# Autodesk Inventor assembly: CycloidalGearBoxAssemblyV2
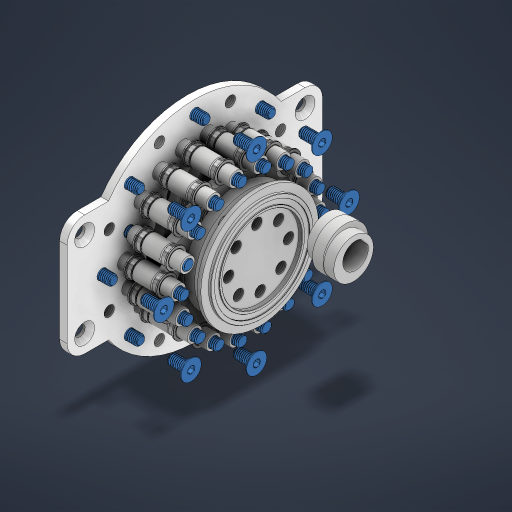
[picture p0: Inventor's stored thumbnail of the model, 512x512]
Saved by Autodesk Inventor 2024 (Build 280153000, 153)
## iProperties
Created: 2024-01-31
Part Number: CycloidalGearBoxAssemblyV2
Document SubType Name: Assembly
Designer: avsar
Author: avsar
## Documents named in this file (20)
- C:\Users\avsar\Documents\Inventor\RCR_Arm\Arm_V4\CycloidalGearBoxes\StageOneGearBox\CycloidalGearBoxAssemblyV2.iam
- C:\Users\avsar\Documents\Inventor\RCR_Arm\Arm_V4\CycloidalGearBoxes\StageOneGearBox\HousingFaceInput.ipt
- C:\Users\avsar\Documents\Inventor\RCR_Arm\Arm_V4\CycloidalGearBoxes\StageOneGearBox\HousingInputFaceSpacer.ipt
- C:\Users\avsar\Documents\Inventor\RCR_Arm\COTS\Motion\Bearings\Flanged Bearings\4x7x2.5mm Flanged Ball Bearing.ipt
- C:\Users\avsar\Documents\Inventor\RCR_Arm\Arm_V4\CycloidalGearBoxes\StageOneGearBox\RollerBearingShaft.ipt
- C:\Users\avsar\Documents\Inventor\RCR_Arm\Arm_V4\CycloidalGearBoxes\StageOneGearBox\EccentricBearingShaft.ipt
- C:\Users\avsar\Documents\Inventor\RCR_Arm\Arm_V4\CycloidalGearBoxes\StageOneGearBox\CycloidalDisk.ipt
- C:\Users\avsar\Documents\Inventor\RCR_Arm\COTS\Motion\Bearings\Standard Bearings\16mm ID x 22mm OD x 4mm Thickness Ball Bearing.ipt
- C:\Users\avsar\Documents\Inventor\RCR_Arm\Arm_V4\CycloidalGearBoxes\StageOneGearBox\OutputPlateSpacer.ipt
- C:\Users\avsar\Documents\Inventor\RCR_Arm\Arm_V4\CycloidalGearBoxes\StageOneGearBox\OutPutPlate.ipt
- C:\Users\avsar\Documents\Inventor\RCR_Arm\COTS\ISO Standard Hardware\Screws\Sockethead Screws\Buttonhead Screws\M4 x 0.7mm\(M4 x 0.7 x 18) Sockethead Buttonhead Screw.ipt
- C:\Users\avsar\Documents\Inventor\RCR_Arm\Arm_V4\CycloidalGearBoxes\StageOneGearBox\HousingLidSpacer.ipt
- C:\Users\avsar\Documents\Inventor\RCR_Arm\COTS\goBilda\Motion\Bearings\32mm ID Flanged Ball Bearing (39mm OD, 5mm Thickness).ipt
- C:\Users\avsar\Documents\Inventor\RCR_Arm\Arm_V4\CycloidalGearBoxes\StageOneGearBox\Gearbox_MainBody.ipt
- C:\Users\avsar\Documents\Inventor\RCR_Arm\Arm_V4\CycloidalGearBoxes\StageOneGearBox\HousingLid.ipt
- C:\Users\avsar\Documents\Inventor\RCR_Arm\Arm_V4\CycloidalGearBoxes\StageOneGearBox\InputSpacer.ipt
- C:\Users\avsar\Documents\Inventor\RCR_Arm\COTS\Motion\Bearings\Flanged Bearings\10x15x4mm Flanged Bearing.ipt
- C:\Users\avsar\Documents\Inventor\RCR_Arm\Arm_V4\CycloidalGearBoxes\StageOneGearBox\OutputBearingDistanceRing.ipt
- C:\Users\avsar\Documents\Inventor\RCR_Arm\COTS\ISO Standard Hardware\Screws\Sockethead Screws\Countersunk Screws\M4 x 0.7mm\(M4 x 0.7 x 8) Sockethead Countersunk Screw.ipt
- C:\Users\avsar\Documents\Inventor\RCR_Arm\Arm_V4\ArmStages\27mm_SandedScrew.ipt
## Components (168 placed, 19 different names)
1. HousingInputFaceSpacer:1 — Mate:3, Mate:4, Mate:305
2. 4x7x2.5mm Flanged Ball Bearing:1 — Mate:3, Mate:4, Mate:5, Mate:6, Mate:13
3. 4x7x2.5mm Flanged Ball Bearing:2 — Mate:7, Mate:8, Mate:108, Mate:109
4. RollerBearingShaft:1 — Mate:5, Mate:6, Mate:7, Mate:8, Mate:287
5. EccentricBearingShaft:1 — Mate:10, Mate:11, Mate:14, Mate:15, Mate:324
6. CycloidalDisk:1 — Flush:1, Mate:9, Mate:13, Mate:25, Tangent:1, Mate:32, Mate:33, Mate:34, Mate:35, Mate:36, Tangent:8, Tangent:9, Tangent:10, Tangent:11, Tangent:12, Tangent:13
7. 16mm ID x 22mm OD x 4mm Thickness Ball Bearing:1 — Flush:1, Mate:9, Mate:10, Mate:11
8. 16mm ID x 22mm OD x 4mm Thickness Ball Bearing:2 — Mate:14, Mate:15, Flush:2, Mate:16
9. CycloidalDisk:2 — Flush:2, Mate:16, Mate:26, Tangent:2, Mate:27, Tangent:3, Mate:28, Tangent:4, Mate:29, Tangent:5, Mate:30, Tangent:6, Mate:31, Tangent:7
10. HousingInputFaceSpacer:2 — Mate:23, Mate:24, Mate:286
11. 4x7x2.5mm Flanged Ball Bearing:3 — Mate:282
12. 4x7x2.5mm Flanged Ball Bearing:4 — Mate:23
13. RollerBearingShaft:2 — Mate:24, Mate:283
14. 4x7x2.5mm Flanged Ball Bearing:5 — Mate:25, Tangent:1, Tangent:12, Mate:66, Mate:89, Mate:96
15. 4x7x2.5mm Flanged Ball Bearing:6 — Mate:28, Tangent:4, Mate:39, Mate:40, Mate:50, Mate:51
16. 4x7x2.5mm Flanged Ball Bearing:7 — Mate:27, Tangent:3, Mate:37, Mate:38
17. 4x7x2.5mm Flanged Ball Bearing:8 — Mate:30, Tangent:6, Mate:43, Mate:44
18. 4x7x2.5mm Flanged Ball Bearing:9 — Mate:31, Tangent:7, Mate:45, Mate:46, Mate:54
19. 4x7x2.5mm Flanged Ball Bearing:10 — Mate:26, Tangent:2, Mate:47, Mate:48, Mate:55
20. 4x7x2.5mm Flanged Ball Bearing:11 — Mate:29, Tangent:5, Mate:41, Mate:42
21. 4x7x2.5mm Flanged Ball Bearing:12 — Mate:32, Tangent:9, Mate:69, Mate:85
22. 4x7x2.5mm Flanged Ball Bearing:13 — Mate:35, Tangent:11, Mate:84, Mate:88, Mate:91
23. 4x7x2.5mm Flanged Ball Bearing:14 — Mate:36, Tangent:8, Mate:57, Mate:58
24. 4x7x2.5mm Flanged Ball Bearing:15 — Mate:33, Tangent:10, Mate:73, Mate:86, Mate:102
25. 4x7x2.5mm Flanged Ball Bearing:16 — Mate:34, Tangent:13, Mate:79, Mate:87, Mate:94
26. OutputPlateSpacer:1 — Mate:37, Mate:38, Mate:49, Mate:56
27. OutPutPlate:1 — Mate:49, Mate:50, Mate:51, Mate:52, Mate:53, Mate:54, Mate:55, Mate:56, Mate:92, Mate:103, Mate:104, Mate:105, Mate:106, Mate:107, Mate:328
28. OutputPlateSpacer:2 — Mate:39, Mate:40
29. OutputPlateSpacer:3 — Mate:41, Mate:42, Mate:52
30. OutputPlateSpacer:4 — Mate:43, Mate:44, Mate:53
31. OutputPlateSpacer:5 — Mate:45, Mate:46
32. OutputPlateSpacer:6 — Mate:47, Mate:48
33. OutputPlateSpacer:7 — Mate:57, Mate:58, Mate:97, Mate:98
34. OutputPlateSpacer:8 — Mate:69, Mate:85, Mate:99, Mate:100
35. OutputPlateSpacer:9 — Mate:66, Mate:89, Mate:95
36. OutputPlateSpacer:10 — Mate:73, Mate:86, Mate:101
37. OutputPlateSpacer:11 — Mate:79, Mate:87, Mate:93
38. OutputPlateSpacer:12 — Mate:84, Mate:88, Mate:90
39. (M4 x 0.7 x 18) Sockethead Buttonhead Screw:1 — Mate:90, Mate:91, Mate:92
40. (M4 x 0.7 x 18) Sockethead Buttonhead Screw:2 — Mate:99, Mate:100, Mate:105
41. (M4 x 0.7 x 18) Sockethead Buttonhead Screw:3 — Mate:97, Mate:98, Mate:104
42. (M4 x 0.7 x 18) Sockethead Buttonhead Screw:4 — Mate:95, Mate:96, Mate:103
43. (M4 x 0.7 x 18) Sockethead Buttonhead Screw:5 — Mate:101, Mate:102, Mate:106
44. (M4 x 0.7 x 18) Sockethead Buttonhead Screw:6 — Mate:93, Mate:94, Mate:107
45. HousingLidSpacer:1 — Mate:108, Mate:109, Flush:3
46. Gearbox_MainBody:1 — Mate:318, Mate:319, Mate:320, Mate:321, Mate:323
47. InputSpacer:1 — Mate:120, Mate:121
48. 10x15x4mm Flanged Bearing:1 — Mate:120, Mate:121, Mate:290, Mate:291, Mate:324
49. HousingInputFaceSpacer:3 — Mate:284, Mate:285
50. 4x7x2.5mm Flanged Ball Bearing:17
51. 4x7x2.5mm Flanged Ball Bearing:18
52. RollerBearingShaft:3
53. HousingLidSpacer:2
54. HousingInputFaceSpacer:4 — Mate:288
55. 4x7x2.5mm Flanged Ball Bearing:19
56. 4x7x2.5mm Flanged Ball Bearing:20
57. RollerBearingShaft:4
58. HousingLidSpacer:3 — Flush:3, Flush:4
59. HousingInputFaceSpacer:5 — Mate:289
60. 4x7x2.5mm Flanged Ball Bearing:21
61. 4x7x2.5mm Flanged Ball Bearing:22
62. RollerBearingShaft:5
63. HousingLidSpacer:4 — Flush:4, Flush:5
64. HousingInputFaceSpacer:6
65. 4x7x2.5mm Flanged Ball Bearing:23
66. 4x7x2.5mm Flanged Ball Bearing:24
67. RollerBearingShaft:6 — Mate:294
68. HousingLidSpacer:5 — Flush:5, Flush:6
69. HousingInputFaceSpacer:7 — Mate:304
70. 4x7x2.5mm Flanged Ball Bearing:25
71. 4x7x2.5mm Flanged Ball Bearing:26
72. RollerBearingShaft:7
73. HousingLidSpacer:6 — Flush:16
74. HousingInputFaceSpacer:8
75. 4x7x2.5mm Flanged Ball Bearing:27
76. 4x7x2.5mm Flanged Ball Bearing:28
77. RollerBearingShaft:8 — Mate:293
78. HousingLidSpacer:7 — Flush:7, Flush:8
79. HousingInputFaceSpacer:9 — Mate:296
80. 4x7x2.5mm Flanged Ball Bearing:29
81. 4x7x2.5mm Flanged Ball Bearing:30
82. RollerBearingShaft:9
83. HousingLidSpacer:8 — Flush:9, Flush:10
84. HousingInputFaceSpacer:10
85. 4x7x2.5mm Flanged Ball Bearing:31
86. 4x7x2.5mm Flanged Ball Bearing:32
87. RollerBearingShaft:10 — Mate:301
88. HousingLidSpacer:9 — Flush:14
89. HousingInputFaceSpacer:11
90. 4x7x2.5mm Flanged Ball Bearing:33
91. 4x7x2.5mm Flanged Ball Bearing:34
92. RollerBearingShaft:11 — Mate:292
93. HousingLidSpacer:10 — Flush:6, Flush:7
94. HousingInputFaceSpacer:12 — Mate:297
95. 4x7x2.5mm Flanged Ball Bearing:35
96. 4x7x2.5mm Flanged Ball Bearing:36
97. RollerBearingShaft:12
98. HousingLidSpacer:11 — Flush:10, Flush:11
99. HousingInputFaceSpacer:13 — Mate:300
100. 4x7x2.5mm Flanged Ball Bearing:37
101. 4x7x2.5mm Flanged Ball Bearing:38
102. RollerBearingShaft:13
103. HousingLidSpacer:12 — Flush:13, Flush:14
104. HousingInputFaceSpacer:14
105. 4x7x2.5mm Flanged Ball Bearing:39
106. 4x7x2.5mm Flanged Ball Bearing:40
107. RollerBearingShaft:14 — Mate:295
108. HousingLidSpacer:13 — Flush:8, Flush:9
109. HousingInputFaceSpacer:15 — Mate:303
110. 4x7x2.5mm Flanged Ball Bearing:41
111. 4x7x2.5mm Flanged Ball Bearing:42
112. RollerBearingShaft:15
113. HousingLidSpacer:14 — Flush:15, Flush:16
114. HousingInputFaceSpacer:17 — Flush:11, Flush:12
115. 4x7x2.5mm Flanged Ball Bearing:45
116. 4x7x2.5mm Flanged Ball Bearing:46
117. RollerBearingShaft:17
118. HousingLidSpacer:16 — Mate:298
119. HousingInputFaceSpacer:18 — Flush:12, Flush:13
120. 4x7x2.5mm Flanged Ball Bearing:47
121. 4x7x2.5mm Flanged Ball Bearing:48
122. RollerBearingShaft:18
123. HousingLidSpacer:17 — Mate:299
124. HousingLidSpacer:18 — Mate:282, Mate:283
125. HousingLid:1 — Mate:318, Mate:322, Mate:323, Mate:325, Mate:326, Flush:34, Mate:348, Flush:35, Mate:349, Flush:36, Mate:350, Flush:37, Mate:351, Flush:38, Mate:352, Flush:39, Mate:353, Flush:40, Mate:354, Flush:41, Mate:355
126. HousingFaceInput:1 — Mate:284, Mate:285, Mate:286, Mate:287, Mate:288, Mate:289, Mate:290, Mate:291, Mate:292, Mate:293, Mate:294, Mate:295, Mate:296, Mate:297, Mate:298, Mate:299, Mate:300, Mate:301, Mate:303, Mate:304, Mate:305, Mate:314, Mate:315, Mate:319, Mate:320, Mate:321, Mate:322, Flush:42, Mate:356, Flush:43, Mate:357, Flush:44, Mate:358, Flush:45, Mate:359, Flush:46, Mate:360, Flush:47, Mate:361, Flush:48, Mate:362, Flush:49, Mate:363, Flush:50, Mate:364, Flush:51, Mate:365, Flush:52, Mate:366, Flush:53, Mate:367, Flush:54, Mate:368, Flush:55, Mate:369, Flush:56, Mate:370, Flush:57, Mate:371, Flush:58, Mate:372, Flush:59, Mate:373, Flush:60, Mate:374, Flush:61, Mate:375, Flush:62, Mate:376, Flush:63, Mate:377, Flush:64, Mate:378, Flush:65, Mate:379, Flush:66, Mate:380, Flush:67, Mate:381
127. HousingInputFaceSpacer:19 — Mate:314, Mate:315
128. 4x7x2.5mm Flanged Ball Bearing:49
129. 4x7x2.5mm Flanged Ball Bearing:50
130. RollerBearingShaft:19
131. HousingLidSpacer:19 — Flush:15
132. 32mm ID Flanged Ball Bearing (39mm OD, 5mm Thickness):1 — Mate:327, Mate:328
133. OutputBearingDistanceRing:1 — Mate:325, Mate:326, Mate:327
134. (M4 x 0.7 x 8) Sockethead Countersunk Screw:1 — Flush:34, Mate:348
135. (M4 x 0.7 x 8) Sockethead Countersunk Screw:2 — Flush:35, Mate:349
136. (M4 x 0.7 x 8) Sockethead Countersunk Screw:3 — Flush:36, Mate:350
137. (M4 x 0.7 x 8) Sockethead Countersunk Screw:4 — Flush:37, Mate:351
138. (M4 x 0.7 x 8) Sockethead Countersunk Screw:5 — Flush:38, Mate:352
139. (M4 x 0.7 x 8) Sockethead Countersunk Screw:6 — Flush:39, Mate:353
140. (M4 x 0.7 x 8) Sockethead Countersunk Screw:7 — Flush:40, Mate:354
141. (M4 x 0.7 x 8) Sockethead Countersunk Screw:8 — Flush:41, Mate:355
142. (M4 x 0.7 x 8) Sockethead Countersunk Screw:9 — Flush:42, Mate:356
143. (M4 x 0.7 x 8) Sockethead Countersunk Screw:10 — Flush:43, Mate:357
144. (M4 x 0.7 x 8) Sockethead Countersunk Screw:11 — Flush:44, Mate:358
145. (M4 x 0.7 x 8) Sockethead Countersunk Screw:12 — Flush:45, Mate:359
146. (M4 x 0.7 x 8) Sockethead Countersunk Screw:13 — Flush:46, Mate:360
147. (M4 x 0.7 x 8) Sockethead Countersunk Screw:14 — Flush:47, Mate:361
148. (M4 x 0.7 x 8) Sockethead Countersunk Screw:15 — Flush:48, Mate:362
149. (M4 x 0.7 x 8) Sockethead Countersunk Screw:16 — Flush:49, Mate:363
150. 27mm_SandedScrew:1 — Flush:50, Mate:364
151. 27mm_SandedScrew:2 — Flush:51, Mate:365
152. 27mm_SandedScrew:3 — Flush:52, Mate:366
153. 27mm_SandedScrew:4 — Flush:53, Mate:367
154. 27mm_SandedScrew:5 — Flush:54, Mate:368
155. 27mm_SandedScrew:6 — Flush:55, Mate:369
156. 27mm_SandedScrew:7 — Flush:56, Mate:370
157. 27mm_SandedScrew:8 — Flush:57, Mate:371
158. 27mm_SandedScrew:9 — Flush:58, Mate:372
159. 27mm_SandedScrew:10 — Flush:59, Mate:373
160. 27mm_SandedScrew:11 — Flush:60, Mate:374
161. 27mm_SandedScrew:12 — Flush:61, Mate:375
162. 27mm_SandedScrew:13 — Flush:62, Mate:376
163. 27mm_SandedScrew:14 — Flush:63, Mate:377
164. 27mm_SandedScrew:15 — Flush:64, Mate:378
165. 27mm_SandedScrew:16 — Flush:65, Mate:379
166. 27mm_SandedScrew:17 — Flush:66, Mate:380
167. 27mm_SandedScrew:18 — Flush:67, Mate:381
168. EccentricBearingShaft:2
## Relationships (346: Mate 283, Flush 50, Tangent 13)
- Mate:3: HousingInputFaceSpacer:1 ↔ 4x7x2.5mm Flanged Ball Bearing:1
- Mate:4: HousingInputFaceSpacer:1 ↔ 4x7x2.5mm Flanged Ball Bearing:1
- Mate:5: 4x7x2.5mm Flanged Ball Bearing:1 ↔ RollerBearingShaft:1
- Mate:6: 4x7x2.5mm Flanged Ball Bearing:1 ↔ RollerBearingShaft:1
- Mate:7: 4x7x2.5mm Flanged Ball Bearing:2 ↔ RollerBearingShaft:1
- Mate:8: 4x7x2.5mm Flanged Ball Bearing:2 ↔ RollerBearingShaft:1
- Flush:1: CycloidalDisk:1 ↔ 16mm ID x 22mm OD x 4mm Thickness Ball Bearing:1
- Mate:9: CycloidalDisk:1 ↔ 16mm ID x 22mm OD x 4mm Thickness Ball Bearing:1
- Mate:10: EccentricBearingShaft:1 ↔ 16mm ID x 22mm OD x 4mm Thickness Ball Bearing:1
- Mate:11: EccentricBearingShaft:1 ↔ 16mm ID x 22mm OD x 4mm Thickness Ball Bearing:1
- Mate:13: 4x7x2.5mm Flanged Ball Bearing:1 ↔ CycloidalDisk:1
- Mate:14: EccentricBearingShaft:1 ↔ 16mm ID x 22mm OD x 4mm Thickness Ball Bearing:2
- Mate:15: EccentricBearingShaft:1 ↔ 16mm ID x 22mm OD x 4mm Thickness Ball Bearing:2
- Flush:2: 16mm ID x 22mm OD x 4mm Thickness Ball Bearing:2 ↔ CycloidalDisk:2
- Mate:16: 16mm ID x 22mm OD x 4mm Thickness Ball Bearing:2 ↔ CycloidalDisk:2
- [Mate]: 4x7x2.5mm Flanged Ball Bearing:3 ↔ RollerBearingShaft:2
- [Mate]: 4x7x2.5mm Flanged Ball Bearing:3 ↔ RollerBearingShaft:2
- [Mate]: 4x7x2.5mm Flanged Ball Bearing:4 ↔ RollerBearingShaft:2
- [Mate]: 4x7x2.5mm Flanged Ball Bearing:4 ↔ RollerBearingShaft:2
- Mate:23: HousingInputFaceSpacer:2 ↔ 4x7x2.5mm Flanged Ball Bearing:4
- Mate:24: HousingInputFaceSpacer:2 ↔ RollerBearingShaft:2
- Mate:25: CycloidalDisk:1 ↔ 4x7x2.5mm Flanged Ball Bearing:5
- Tangent:1: CycloidalDisk:1 ↔ 4x7x2.5mm Flanged Ball Bearing:5
- Mate:26: CycloidalDisk:2 ↔ 4x7x2.5mm Flanged Ball Bearing:10
- Tangent:2: CycloidalDisk:2 ↔ 4x7x2.5mm Flanged Ball Bearing:10
- Mate:27: CycloidalDisk:2 ↔ 4x7x2.5mm Flanged Ball Bearing:7
- Tangent:3: CycloidalDisk:2 ↔ 4x7x2.5mm Flanged Ball Bearing:7
- Mate:28: CycloidalDisk:2 ↔ 4x7x2.5mm Flanged Ball Bearing:6
- Tangent:4: CycloidalDisk:2 ↔ 4x7x2.5mm Flanged Ball Bearing:6
- Mate:29: CycloidalDisk:2 ↔ 4x7x2.5mm Flanged Ball Bearing:11
- Tangent:5: CycloidalDisk:2 ↔ 4x7x2.5mm Flanged Ball Bearing:11
- Mate:30: CycloidalDisk:2 ↔ 4x7x2.5mm Flanged Ball Bearing:8
- Tangent:6: CycloidalDisk:2 ↔ 4x7x2.5mm Flanged Ball Bearing:8
- Mate:31: CycloidalDisk:2 ↔ 4x7x2.5mm Flanged Ball Bearing:9
- Tangent:7: CycloidalDisk:2 ↔ 4x7x2.5mm Flanged Ball Bearing:9
- Mate:32: CycloidalDisk:1 ↔ 4x7x2.5mm Flanged Ball Bearing:12
- Mate:33: CycloidalDisk:1 ↔ 4x7x2.5mm Flanged Ball Bearing:15
- Mate:34: CycloidalDisk:1 ↔ 4x7x2.5mm Flanged Ball Bearing:16
- Mate:35: CycloidalDisk:1 ↔ 4x7x2.5mm Flanged Ball Bearing:13
- Mate:36: CycloidalDisk:1 ↔ 4x7x2.5mm Flanged Ball Bearing:14
- Tangent:8: CycloidalDisk:1 ↔ 4x7x2.5mm Flanged Ball Bearing:14
- Tangent:9: CycloidalDisk:1 ↔ 4x7x2.5mm Flanged Ball Bearing:12
- Tangent:10: CycloidalDisk:1 ↔ 4x7x2.5mm Flanged Ball Bearing:15
- Tangent:11: CycloidalDisk:1 ↔ 4x7x2.5mm Flanged Ball Bearing:13
- Mate:37: 4x7x2.5mm Flanged Ball Bearing:7 ↔ OutputPlateSpacer:1
- Mate:38: 4x7x2.5mm Flanged Ball Bearing:7 ↔ OutputPlateSpacer:1
- Mate:39: 4x7x2.5mm Flanged Ball Bearing:6 ↔ OutputPlateSpacer:2
- Mate:40: 4x7x2.5mm Flanged Ball Bearing:6 ↔ OutputPlateSpacer:2
- Mate:41: 4x7x2.5mm Flanged Ball Bearing:11 ↔ OutputPlateSpacer:3
- Mate:42: 4x7x2.5mm Flanged Ball Bearing:11 ↔ OutputPlateSpacer:3
- Mate:43: 4x7x2.5mm Flanged Ball Bearing:8 ↔ OutputPlateSpacer:4
- Mate:44: 4x7x2.5mm Flanged Ball Bearing:8 ↔ OutputPlateSpacer:4
- Mate:45: 4x7x2.5mm Flanged Ball Bearing:9 ↔ OutputPlateSpacer:5
- Mate:46: 4x7x2.5mm Flanged Ball Bearing:9 ↔ OutputPlateSpacer:5
- Mate:47: 4x7x2.5mm Flanged Ball Bearing:10 ↔ OutputPlateSpacer:6
- Mate:48: 4x7x2.5mm Flanged Ball Bearing:10 ↔ OutputPlateSpacer:6
- Mate:49: OutputPlateSpacer:1 ↔ OutPutPlate:1
- Mate:50: 4x7x2.5mm Flanged Ball Bearing:6 ↔ OutPutPlate:1
- Mate:51: 4x7x2.5mm Flanged Ball Bearing:6 ↔ OutPutPlate:1
- Mate:52: OutPutPlate:1 ↔ OutputPlateSpacer:3
- Mate:53: OutPutPlate:1 ↔ OutputPlateSpacer:4
- Mate:54: 4x7x2.5mm Flanged Ball Bearing:9 ↔ OutPutPlate:1
- Mate:55: 4x7x2.5mm Flanged Ball Bearing:10 ↔ OutPutPlate:1
- Mate:56: OutputPlateSpacer:1 ↔ OutPutPlate:1
- Mate:57: 4x7x2.5mm Flanged Ball Bearing:14 ↔ OutputPlateSpacer:7
- Mate:58: 4x7x2.5mm Flanged Ball Bearing:14 ↔ OutputPlateSpacer:7
- Tangent:12: CycloidalDisk:1 ↔ 4x7x2.5mm Flanged Ball Bearing:5
- Tangent:13: CycloidalDisk:1 ↔ 4x7x2.5mm Flanged Ball Bearing:16
- Mate:66: 4x7x2.5mm Flanged Ball Bearing:5 ↔ OutputPlateSpacer:9
- Mate:69: 4x7x2.5mm Flanged Ball Bearing:12 ↔ OutputPlateSpacer:8
- Mate:73: 4x7x2.5mm Flanged Ball Bearing:15 ↔ OutputPlateSpacer:10
- Mate:79: 4x7x2.5mm Flanged Ball Bearing:16 ↔ OutputPlateSpacer:11
- Mate:84: 4x7x2.5mm Flanged Ball Bearing:13 ↔ OutputPlateSpacer:12
- Mate:85: 4x7x2.5mm Flanged Ball Bearing:12 ↔ OutputPlateSpacer:8
- Mate:86: 4x7x2.5mm Flanged Ball Bearing:15 ↔ OutputPlateSpacer:10
- Mate:87: 4x7x2.5mm Flanged Ball Bearing:16 ↔ OutputPlateSpacer:11
- Mate:88: 4x7x2.5mm Flanged Ball Bearing:13 ↔ OutputPlateSpacer:12
- Mate:89: 4x7x2.5mm Flanged Ball Bearing:5 ↔ OutputPlateSpacer:9
- Mate:90: OutputPlateSpacer:12 ↔ (M4 x 0.7 x 18) Sockethead Buttonhead Screw:1
- Mate:91: 4x7x2.5mm Flanged Ball Bearing:13 ↔ (M4 x 0.7 x 18) Sockethead Buttonhead Screw:1
- Mate:92: OutPutPlate:1 ↔ (M4 x 0.7 x 18) Sockethead Buttonhead Screw:1
- Mate:93: OutputPlateSpacer:11 ↔ (M4 x 0.7 x 18) Sockethead Buttonhead Screw:6
- Mate:94: 4x7x2.5mm Flanged Ball Bearing:16 ↔ (M4 x 0.7 x 18) Sockethead Buttonhead Screw:6
- Mate:95: OutputPlateSpacer:9 ↔ (M4 x 0.7 x 18) Sockethead Buttonhead Screw:4
- Mate:96: 4x7x2.5mm Flanged Ball Bearing:5 ↔ (M4 x 0.7 x 18) Sockethead Buttonhead Screw:4
- Mate:97: OutputPlateSpacer:7 ↔ (M4 x 0.7 x 18) Sockethead Buttonhead Screw:3
- Mate:98: OutputPlateSpacer:7 ↔ (M4 x 0.7 x 18) Sockethead Buttonhead Screw:3
- Mate:99: OutputPlateSpacer:8 ↔ (M4 x 0.7 x 18) Sockethead Buttonhead Screw:2
- Mate:100: OutputPlateSpacer:8 ↔ (M4 x 0.7 x 18) Sockethead Buttonhead Screw:2
- Mate:101: OutputPlateSpacer:10 ↔ (M4 x 0.7 x 18) Sockethead Buttonhead Screw:5
- Mate:102: 4x7x2.5mm Flanged Ball Bearing:15 ↔ (M4 x 0.7 x 18) Sockethead Buttonhead Screw:5
- Mate:103: OutPutPlate:1 ↔ (M4 x 0.7 x 18) Sockethead Buttonhead Screw:4
- Mate:104: OutPutPlate:1 ↔ (M4 x 0.7 x 18) Sockethead Buttonhead Screw:3
- Mate:105: OutPutPlate:1 ↔ (M4 x 0.7 x 18) Sockethead Buttonhead Screw:2
- Mate:106: OutPutPlate:1 ↔ (M4 x 0.7 x 18) Sockethead Buttonhead Screw:5
- Mate:107: OutPutPlate:1 ↔ (M4 x 0.7 x 18) Sockethead Buttonhead Screw:6
- Mate:108: 4x7x2.5mm Flanged Ball Bearing:2 ↔ HousingLidSpacer:1
- Mate:109: 4x7x2.5mm Flanged Ball Bearing:2 ↔ HousingLidSpacer:1
- Mate:120: InputSpacer:1 ↔ 10x15x4mm Flanged Bearing:1
- Mate:121: InputSpacer:1 ↔ 10x15x4mm Flanged Bearing:1
- [Mate]: HousingInputFaceSpacer:3 ↔ 4x7x2.5mm Flanged Ball Bearing:17
- [Mate]: HousingInputFaceSpacer:3 ↔ 4x7x2.5mm Flanged Ball Bearing:17
- [Mate]: 4x7x2.5mm Flanged Ball Bearing:17 ↔ RollerBearingShaft:3
- [Mate]: 4x7x2.5mm Flanged Ball Bearing:17 ↔ RollerBearingShaft:3
- [Mate]: 4x7x2.5mm Flanged Ball Bearing:18 ↔ RollerBearingShaft:3
- [Mate]: 4x7x2.5mm Flanged Ball Bearing:18 ↔ RollerBearingShaft:3
- [Mate]: 4x7x2.5mm Flanged Ball Bearing:18 ↔ HousingLidSpacer:2
- [Mate]: 4x7x2.5mm Flanged Ball Bearing:18 ↔ HousingLidSpacer:2
- [Mate]: HousingInputFaceSpacer:4 ↔ 4x7x2.5mm Flanged Ball Bearing:19
- [Mate]: HousingInputFaceSpacer:4 ↔ 4x7x2.5mm Flanged Ball Bearing:19
- [Mate]: 4x7x2.5mm Flanged Ball Bearing:19 ↔ RollerBearingShaft:4
- [Mate]: 4x7x2.5mm Flanged Ball Bearing:19 ↔ RollerBearingShaft:4
- [Mate]: 4x7x2.5mm Flanged Ball Bearing:20 ↔ RollerBearingShaft:4
- [Mate]: 4x7x2.5mm Flanged Ball Bearing:20 ↔ RollerBearingShaft:4
- [Mate]: 4x7x2.5mm Flanged Ball Bearing:20 ↔ HousingLidSpacer:3
- [Mate]: 4x7x2.5mm Flanged Ball Bearing:20 ↔ HousingLidSpacer:3
- [Mate]: HousingInputFaceSpacer:5 ↔ 4x7x2.5mm Flanged Ball Bearing:21
- [Mate]: HousingInputFaceSpacer:5 ↔ 4x7x2.5mm Flanged Ball Bearing:21
- [Mate]: 4x7x2.5mm Flanged Ball Bearing:21 ↔ RollerBearingShaft:5
- [Mate]: 4x7x2.5mm Flanged Ball Bearing:21 ↔ RollerBearingShaft:5
- [Mate]: 4x7x2.5mm Flanged Ball Bearing:22 ↔ RollerBearingShaft:5
- [Mate]: 4x7x2.5mm Flanged Ball Bearing:22 ↔ RollerBearingShaft:5
- [Mate]: 4x7x2.5mm Flanged Ball Bearing:22 ↔ HousingLidSpacer:4
- [Mate]: 4x7x2.5mm Flanged Ball Bearing:22 ↔ HousingLidSpacer:4
- [Mate]: HousingInputFaceSpacer:6 ↔ 4x7x2.5mm Flanged Ball Bearing:23
- [Mate]: HousingInputFaceSpacer:6 ↔ 4x7x2.5mm Flanged Ball Bearing:23
- [Mate]: 4x7x2.5mm Flanged Ball Bearing:23 ↔ RollerBearingShaft:6
- [Mate]: 4x7x2.5mm Flanged Ball Bearing:23 ↔ RollerBearingShaft:6
- [Mate]: 4x7x2.5mm Flanged Ball Bearing:24 ↔ RollerBearingShaft:6
- [Mate]: 4x7x2.5mm Flanged Ball Bearing:24 ↔ RollerBearingShaft:6
- [Mate]: 4x7x2.5mm Flanged Ball Bearing:24 ↔ HousingLidSpacer:5
- [Mate]: 4x7x2.5mm Flanged Ball Bearing:24 ↔ HousingLidSpacer:5
- [Mate]: HousingInputFaceSpacer:7 ↔ 4x7x2.5mm Flanged Ball Bearing:25
- [Mate]: HousingInputFaceSpacer:7 ↔ 4x7x2.5mm Flanged Ball Bearing:25
- [Mate]: 4x7x2.5mm Flanged Ball Bearing:25 ↔ RollerBearingShaft:7
- [Mate]: 4x7x2.5mm Flanged Ball Bearing:25 ↔ RollerBearingShaft:7
- [Mate]: 4x7x2.5mm Flanged Ball Bearing:26 ↔ RollerBearingShaft:7
- [Mate]: 4x7x2.5mm Flanged Ball Bearing:26 ↔ RollerBearingShaft:7
- [Mate]: 4x7x2.5mm Flanged Ball Bearing:26 ↔ HousingLidSpacer:6
- [Mate]: 4x7x2.5mm Flanged Ball Bearing:26 ↔ HousingLidSpacer:6
- [Mate]: HousingInputFaceSpacer:8 ↔ 4x7x2.5mm Flanged Ball Bearing:27
- [Mate]: HousingInputFaceSpacer:8 ↔ 4x7x2.5mm Flanged Ball Bearing:27
- [Mate]: 4x7x2.5mm Flanged Ball Bearing:27 ↔ RollerBearingShaft:8
- [Mate]: 4x7x2.5mm Flanged Ball Bearing:27 ↔ RollerBearingShaft:8
- [Mate]: 4x7x2.5mm Flanged Ball Bearing:28 ↔ RollerBearingShaft:8
- [Mate]: 4x7x2.5mm Flanged Ball Bearing:28 ↔ RollerBearingShaft:8
- [Mate]: 4x7x2.5mm Flanged Ball Bearing:28 ↔ HousingLidSpacer:7
- [Mate]: 4x7x2.5mm Flanged Ball Bearing:28 ↔ HousingLidSpacer:7
- [Mate]: HousingInputFaceSpacer:9 ↔ 4x7x2.5mm Flanged Ball Bearing:29
- [Mate]: HousingInputFaceSpacer:9 ↔ 4x7x2.5mm Flanged Ball Bearing:29
- [Mate]: 4x7x2.5mm Flanged Ball Bearing:29 ↔ RollerBearingShaft:9
- [Mate]: 4x7x2.5mm Flanged Ball Bearing:29 ↔ RollerBearingShaft:9
- [Mate]: 4x7x2.5mm Flanged Ball Bearing:30 ↔ RollerBearingShaft:9
- [Mate]: 4x7x2.5mm Flanged Ball Bearing:30 ↔ RollerBearingShaft:9
- [Mate]: 4x7x2.5mm Flanged Ball Bearing:30 ↔ HousingLidSpacer:8
- [Mate]: 4x7x2.5mm Flanged Ball Bearing:30 ↔ HousingLidSpacer:8
- [Mate]: HousingInputFaceSpacer:10 ↔ 4x7x2.5mm Flanged Ball Bearing:31
- [Mate]: HousingInputFaceSpacer:10 ↔ 4x7x2.5mm Flanged Ball Bearing:31
- [Mate]: 4x7x2.5mm Flanged Ball Bearing:31 ↔ RollerBearingShaft:10
- [Mate]: 4x7x2.5mm Flanged Ball Bearing:31 ↔ RollerBearingShaft:10
- [Mate]: 4x7x2.5mm Flanged Ball Bearing:32 ↔ RollerBearingShaft:10
- [Mate]: 4x7x2.5mm Flanged Ball Bearing:32 ↔ RollerBearingShaft:10
- [Mate]: 4x7x2.5mm Flanged Ball Bearing:32 ↔ HousingLidSpacer:9
- [Mate]: 4x7x2.5mm Flanged Ball Bearing:32 ↔ HousingLidSpacer:9
- [Mate]: HousingInputFaceSpacer:11 ↔ 4x7x2.5mm Flanged Ball Bearing:33
- [Mate]: HousingInputFaceSpacer:11 ↔ 4x7x2.5mm Flanged Ball Bearing:33
- [Mate]: 4x7x2.5mm Flanged Ball Bearing:33 ↔ RollerBearingShaft:11
- [Mate]: 4x7x2.5mm Flanged Ball Bearing:33 ↔ RollerBearingShaft:11
- [Mate]: 4x7x2.5mm Flanged Ball Bearing:34 ↔ RollerBearingShaft:11
- [Mate]: 4x7x2.5mm Flanged Ball Bearing:34 ↔ RollerBearingShaft:11
- [Mate]: 4x7x2.5mm Flanged Ball Bearing:34 ↔ HousingLidSpacer:10
- [Mate]: 4x7x2.5mm Flanged Ball Bearing:34 ↔ HousingLidSpacer:10
- [Mate]: HousingInputFaceSpacer:12 ↔ 4x7x2.5mm Flanged Ball Bearing:35
- [Mate]: HousingInputFaceSpacer:12 ↔ 4x7x2.5mm Flanged Ball Bearing:35
- [Mate]: 4x7x2.5mm Flanged Ball Bearing:35 ↔ RollerBearingShaft:12
- [Mate]: 4x7x2.5mm Flanged Ball Bearing:35 ↔ RollerBearingShaft:12
- [Mate]: 4x7x2.5mm Flanged Ball Bearing:36 ↔ RollerBearingShaft:12
- [Mate]: 4x7x2.5mm Flanged Ball Bearing:36 ↔ RollerBearingShaft:12
- [Mate]: 4x7x2.5mm Flanged Ball Bearing:36 ↔ HousingLidSpacer:11
- [Mate]: 4x7x2.5mm Flanged Ball Bearing:36 ↔ HousingLidSpacer:11
- [Mate]: HousingInputFaceSpacer:13 ↔ 4x7x2.5mm Flanged Ball Bearing:37
- [Mate]: HousingInputFaceSpacer:13 ↔ 4x7x2.5mm Flanged Ball Bearing:37
- [Mate]: 4x7x2.5mm Flanged Ball Bearing:37 ↔ RollerBearingShaft:13
- [Mate]: 4x7x2.5mm Flanged Ball Bearing:37 ↔ RollerBearingShaft:13
- [Mate]: 4x7x2.5mm Flanged Ball Bearing:38 ↔ RollerBearingShaft:13
- [Mate]: 4x7x2.5mm Flanged Ball Bearing:38 ↔ RollerBearingShaft:13
- [Mate]: 4x7x2.5mm Flanged Ball Bearing:38 ↔ HousingLidSpacer:12
- [Mate]: 4x7x2.5mm Flanged Ball Bearing:38 ↔ HousingLidSpacer:12
- [Mate]: HousingInputFaceSpacer:14 ↔ 4x7x2.5mm Flanged Ball Bearing:39
- [Mate]: HousingInputFaceSpacer:14 ↔ 4x7x2.5mm Flanged Ball Bearing:39
- [Mate]: 4x7x2.5mm Flanged Ball Bearing:39 ↔ RollerBearingShaft:14
- [Mate]: 4x7x2.5mm Flanged Ball Bearing:39 ↔ RollerBearingShaft:14
- [Mate]: 4x7x2.5mm Flanged Ball Bearing:40 ↔ RollerBearingShaft:14
- [Mate]: 4x7x2.5mm Flanged Ball Bearing:40 ↔ RollerBearingShaft:14
- [Mate]: 4x7x2.5mm Flanged Ball Bearing:40 ↔ HousingLidSpacer:13
- [Mate]: 4x7x2.5mm Flanged Ball Bearing:40 ↔ HousingLidSpacer:13
- [Mate]: HousingInputFaceSpacer:15 ↔ 4x7x2.5mm Flanged Ball Bearing:41
- [Mate]: HousingInputFaceSpacer:15 ↔ 4x7x2.5mm Flanged Ball Bearing:41
- [Mate]: 4x7x2.5mm Flanged Ball Bearing:41 ↔ RollerBearingShaft:15
- [Mate]: 4x7x2.5mm Flanged Ball Bearing:41 ↔ RollerBearingShaft:15
- [Mate]: 4x7x2.5mm Flanged Ball Bearing:42 ↔ RollerBearingShaft:15
- [Mate]: 4x7x2.5mm Flanged Ball Bearing:42 ↔ RollerBearingShaft:15
- [Mate]: 4x7x2.5mm Flanged Ball Bearing:42 ↔ HousingLidSpacer:14
- [Mate]: 4x7x2.5mm Flanged Ball Bearing:42 ↔ HousingLidSpacer:14
- [Mate]: HousingInputFaceSpacer:17 ↔ 4x7x2.5mm Flanged Ball Bearing:45
- [Mate]: HousingInputFaceSpacer:17 ↔ 4x7x2.5mm Flanged Ball Bearing:45
- [Mate]: 4x7x2.5mm Flanged Ball Bearing:45 ↔ RollerBearingShaft:17
- [Mate]: 4x7x2.5mm Flanged Ball Bearing:45 ↔ RollerBearingShaft:17
- [Mate]: 4x7x2.5mm Flanged Ball Bearing:46 ↔ RollerBearingShaft:17
- [Mate]: 4x7x2.5mm Flanged Ball Bearing:46 ↔ RollerBearingShaft:17
- [Mate]: 4x7x2.5mm Flanged Ball Bearing:46 ↔ HousingLidSpacer:16
- [Mate]: 4x7x2.5mm Flanged Ball Bearing:46 ↔ HousingLidSpacer:16
- [Mate]: HousingInputFaceSpacer:18 ↔ 4x7x2.5mm Flanged Ball Bearing:47
- [Mate]: HousingInputFaceSpacer:18 ↔ 4x7x2.5mm Flanged Ball Bearing:47
- [Mate]: 4x7x2.5mm Flanged Ball Bearing:47 ↔ RollerBearingShaft:18
- [Mate]: 4x7x2.5mm Flanged Ball Bearing:47 ↔ RollerBearingShaft:18
- [Mate]: 4x7x2.5mm Flanged Ball Bearing:48 ↔ RollerBearingShaft:18
- [Mate]: 4x7x2.5mm Flanged Ball Bearing:48 ↔ RollerBearingShaft:18
- [Mate]: 4x7x2.5mm Flanged Ball Bearing:48 ↔ HousingLidSpacer:17
- [Mate]: 4x7x2.5mm Flanged Ball Bearing:48 ↔ HousingLidSpacer:17
- Mate:282: 4x7x2.5mm Flanged Ball Bearing:3 ↔ HousingLidSpacer:18
- Mate:283: RollerBearingShaft:2 ↔ HousingLidSpacer:18
- Mate:284: HousingInputFaceSpacer:3 ↔ HousingFaceInput:1
- Mate:285: HousingInputFaceSpacer:3 ↔ HousingFaceInput:1
- Mate:286: HousingInputFaceSpacer:2 ↔ HousingFaceInput:1
- Mate:287: RollerBearingShaft:1 ↔ HousingFaceInput:1
- Mate:288: HousingInputFaceSpacer:4 ↔ HousingFaceInput:1
- Mate:289: HousingInputFaceSpacer:5 ↔ HousingFaceInput:1
- Mate:290: 10x15x4mm Flanged Bearing:1 ↔ HousingFaceInput:1
- Mate:291: 10x15x4mm Flanged Bearing:1 ↔ HousingFaceInput:1
- Mate:292: RollerBearingShaft:11 ↔ HousingFaceInput:1
- Mate:293: RollerBearingShaft:8 ↔ HousingFaceInput:1
- Mate:294: RollerBearingShaft:6 ↔ HousingFaceInput:1
- Mate:295: RollerBearingShaft:14 ↔ HousingFaceInput:1
- Mate:296: HousingInputFaceSpacer:9 ↔ HousingFaceInput:1
- Mate:297: HousingInputFaceSpacer:12 ↔ HousingFaceInput:1
- Mate:298: HousingLidSpacer:16 ↔ HousingFaceInput:1
- Mate:299: HousingLidSpacer:17 ↔ HousingFaceInput:1
- Mate:300: HousingInputFaceSpacer:13 ↔ HousingFaceInput:1
- Mate:301: RollerBearingShaft:10 ↔ HousingFaceInput:1
- Mate:303: HousingInputFaceSpacer:15 ↔ HousingFaceInput:1
- Mate:304: HousingInputFaceSpacer:7 ↔ HousingFaceInput:1
- Mate:305: HousingInputFaceSpacer:1 ↔ HousingFaceInput:1
- Flush:3: HousingLidSpacer:1 ↔ HousingLidSpacer:3
- Flush:4: HousingLidSpacer:3 ↔ HousingLidSpacer:4
- Flush:5: HousingLidSpacer:4 ↔ HousingLidSpacer:5
- Flush:6: HousingLidSpacer:5 ↔ HousingLidSpacer:10
- Flush:7: HousingLidSpacer:7 ↔ HousingLidSpacer:10
- Flush:8: HousingLidSpacer:7 ↔ HousingLidSpacer:13
- Flush:9: HousingLidSpacer:8 ↔ HousingLidSpacer:13
- Flush:10: HousingLidSpacer:8 ↔ HousingLidSpacer:11
- Flush:11: HousingLidSpacer:11 ↔ HousingInputFaceSpacer:17
- Flush:12: HousingInputFaceSpacer:17 ↔ HousingInputFaceSpacer:18
- Flush:13: HousingLidSpacer:12 ↔ HousingInputFaceSpacer:18
- Flush:14: HousingLidSpacer:9 ↔ HousingLidSpacer:12
- [Mate]: HousingInputFaceSpacer:19 ↔ 4x7x2.5mm Flanged Ball Bearing:49
- [Mate]: HousingInputFaceSpacer:19 ↔ 4x7x2.5mm Flanged Ball Bearing:49
- [Mate]: 4x7x2.5mm Flanged Ball Bearing:49 ↔ RollerBearingShaft:19
- [Mate]: 4x7x2.5mm Flanged Ball Bearing:49 ↔ RollerBearingShaft:19
- [Mate]: 4x7x2.5mm Flanged Ball Bearing:50 ↔ RollerBearingShaft:19
- [Mate]: 4x7x2.5mm Flanged Ball Bearing:50 ↔ RollerBearingShaft:19
- [Mate]: 4x7x2.5mm Flanged Ball Bearing:50 ↔ HousingLidSpacer:19
- [Mate]: 4x7x2.5mm Flanged Ball Bearing:50 ↔ HousingLidSpacer:19
- Mate:314: HousingFaceInput:1 ↔ HousingInputFaceSpacer:19
- Mate:315: HousingFaceInput:1 ↔ HousingInputFaceSpacer:19
- Flush:15: HousingLidSpacer:14 ↔ HousingLidSpacer:19
- Flush:16: HousingLidSpacer:6 ↔ HousingLidSpacer:14
- Mate:318: Gearbox_MainBody:1 ↔ HousingLid:1
- Mate:319: Gearbox_MainBody:1 ↔ HousingFaceInput:1
- Mate:320: Gearbox_MainBody:1 ↔ HousingFaceInput:1
- Mate:321: Gearbox_MainBody:1 ↔ HousingFaceInput:1
- Mate:322: HousingLid:1 ↔ HousingFaceInput:1
- Mate:323: Gearbox_MainBody:1 ↔ HousingLid:1
- Mate:324: EccentricBearingShaft:1 ↔ 10x15x4mm Flanged Bearing:1
- Mate:325: HousingLid:1 ↔ OutputBearingDistanceRing:1
- Mate:326: HousingLid:1 ↔ OutputBearingDistanceRing:1
- Mate:327: 32mm ID Flanged Ball Bearing (39mm OD, 5mm Thickness):1 ↔ OutputBearingDistanceRing:1
- Mate:328: OutPutPlate:1 ↔ 32mm ID Flanged Ball Bearing (39mm OD, 5mm Thickness):1
- Flush:34 (-0.3 mm): HousingLid:1 ↔ (M4 x 0.7 x 8) Sockethead Countersunk Screw:1
- Mate:348: HousingLid:1 ↔ (M4 x 0.7 x 8) Sockethead Countersunk Screw:1
- Flush:35 (-0.3 mm): HousingLid:1 ↔ (M4 x 0.7 x 8) Sockethead Countersunk Screw:2
- Mate:349: HousingLid:1 ↔ (M4 x 0.7 x 8) Sockethead Countersunk Screw:2
- Flush:36 (-0.3 mm): HousingLid:1 ↔ (M4 x 0.7 x 8) Sockethead Countersunk Screw:3
- Mate:350: HousingLid:1 ↔ (M4 x 0.7 x 8) Sockethead Countersunk Screw:3
- Flush:37 (-0.3 mm): HousingLid:1 ↔ (M4 x 0.7 x 8) Sockethead Countersunk Screw:4
- Mate:351: HousingLid:1 ↔ (M4 x 0.7 x 8) Sockethead Countersunk Screw:4
- Flush:38 (-0.3 mm): HousingLid:1 ↔ (M4 x 0.7 x 8) Sockethead Countersunk Screw:5
- Mate:352: HousingLid:1 ↔ (M4 x 0.7 x 8) Sockethead Countersunk Screw:5
- Flush:39 (-0.3 mm): HousingLid:1 ↔ (M4 x 0.7 x 8) Sockethead Countersunk Screw:6
- Mate:353: HousingLid:1 ↔ (M4 x 0.7 x 8) Sockethead Countersunk Screw:6
- Flush:40 (-0.3 mm): HousingLid:1 ↔ (M4 x 0.7 x 8) Sockethead Countersunk Screw:7
- Mate:354: HousingLid:1 ↔ (M4 x 0.7 x 8) Sockethead Countersunk Screw:7
- Flush:41 (-0.3 mm): HousingLid:1 ↔ (M4 x 0.7 x 8) Sockethead Countersunk Screw:8
- Mate:355: HousingLid:1 ↔ (M4 x 0.7 x 8) Sockethead Countersunk Screw:8
- Flush:42 (-0.3 mm): HousingFaceInput:1 ↔ (M4 x 0.7 x 8) Sockethead Countersunk Screw:9
- Mate:356: HousingFaceInput:1 ↔ (M4 x 0.7 x 8) Sockethead Countersunk Screw:9
- Flush:43 (-0.3 mm): HousingFaceInput:1 ↔ (M4 x 0.7 x 8) Sockethead Countersunk Screw:10
- Mate:357: HousingFaceInput:1 ↔ (M4 x 0.7 x 8) Sockethead Countersunk Screw:10
- Flush:44 (-0.3 mm): HousingFaceInput:1 ↔ (M4 x 0.7 x 8) Sockethead Countersunk Screw:11
- Mate:358: HousingFaceInput:1 ↔ (M4 x 0.7 x 8) Sockethead Countersunk Screw:11
- Flush:45 (-0.3 mm): HousingFaceInput:1 ↔ (M4 x 0.7 x 8) Sockethead Countersunk Screw:12
- Mate:359: HousingFaceInput:1 ↔ (M4 x 0.7 x 8) Sockethead Countersunk Screw:12
- Flush:46 (-0.3 mm): HousingFaceInput:1 ↔ (M4 x 0.7 x 8) Sockethead Countersunk Screw:13
- Mate:360: HousingFaceInput:1 ↔ (M4 x 0.7 x 8) Sockethead Countersunk Screw:13
- Flush:47 (-0.3 mm): HousingFaceInput:1 ↔ (M4 x 0.7 x 8) Sockethead Countersunk Screw:14
- Mate:361: HousingFaceInput:1 ↔ (M4 x 0.7 x 8) Sockethead Countersunk Screw:14
- Flush:48 (-0.3 mm): HousingFaceInput:1 ↔ (M4 x 0.7 x 8) Sockethead Countersunk Screw:15
- Mate:362: HousingFaceInput:1 ↔ (M4 x 0.7 x 8) Sockethead Countersunk Screw:15
- Flush:49 (-0.3 mm): HousingFaceInput:1 ↔ (M4 x 0.7 x 8) Sockethead Countersunk Screw:16
- Mate:363: HousingFaceInput:1 ↔ (M4 x 0.7 x 8) Sockethead Countersunk Screw:16
- Flush:50 (-0.3 mm): HousingFaceInput:1 ↔ 27mm_SandedScrew:1
- Mate:364: HousingFaceInput:1 ↔ 27mm_SandedScrew:1
- Flush:51 (-0.3 mm): HousingFaceInput:1 ↔ 27mm_SandedScrew:2
- Mate:365: HousingFaceInput:1 ↔ 27mm_SandedScrew:2
- Flush:52 (-0.3 mm): HousingFaceInput:1 ↔ 27mm_SandedScrew:3
- Mate:366: HousingFaceInput:1 ↔ 27mm_SandedScrew:3
- Flush:53 (-0.3 mm): HousingFaceInput:1 ↔ 27mm_SandedScrew:4
- Mate:367: HousingFaceInput:1 ↔ 27mm_SandedScrew:4
- Flush:54 (-0.3 mm): HousingFaceInput:1 ↔ 27mm_SandedScrew:5
- Mate:368: HousingFaceInput:1 ↔ 27mm_SandedScrew:5
- Flush:55 (-0.3 mm): HousingFaceInput:1 ↔ 27mm_SandedScrew:6
- Mate:369: HousingFaceInput:1 ↔ 27mm_SandedScrew:6
- Flush:56 (-0.3 mm): HousingFaceInput:1 ↔ 27mm_SandedScrew:7
- Mate:370: HousingFaceInput:1 ↔ 27mm_SandedScrew:7
- Flush:57 (-0.3 mm): HousingFaceInput:1 ↔ 27mm_SandedScrew:8
- Mate:371: HousingFaceInput:1 ↔ 27mm_SandedScrew:8
- Flush:58 (-0.3 mm): HousingFaceInput:1 ↔ 27mm_SandedScrew:9
- Mate:372: HousingFaceInput:1 ↔ 27mm_SandedScrew:9
- Flush:59 (-0.3 mm): HousingFaceInput:1 ↔ 27mm_SandedScrew:10
- Mate:373: HousingFaceInput:1 ↔ 27mm_SandedScrew:10
- Flush:60 (-0.3 mm): HousingFaceInput:1 ↔ 27mm_SandedScrew:11
- Mate:374: HousingFaceInput:1 ↔ 27mm_SandedScrew:11
- Flush:61 (-0.3 mm): HousingFaceInput:1 ↔ 27mm_SandedScrew:12
- Mate:375: HousingFaceInput:1 ↔ 27mm_SandedScrew:12
- Flush:62 (-0.3 mm): HousingFaceInput:1 ↔ 27mm_SandedScrew:13
- Mate:376: HousingFaceInput:1 ↔ 27mm_SandedScrew:13
- Flush:63 (-0.3 mm): HousingFaceInput:1 ↔ 27mm_SandedScrew:14
- Mate:377: HousingFaceInput:1 ↔ 27mm_SandedScrew:14
- Flush:64 (-0.3 mm): HousingFaceInput:1 ↔ 27mm_SandedScrew:15
- Mate:378: HousingFaceInput:1 ↔ 27mm_SandedScrew:15
- Flush:65 (-0.3 mm): HousingFaceInput:1 ↔ 27mm_SandedScrew:16
- Mate:379: HousingFaceInput:1 ↔ 27mm_SandedScrew:16
- Flush:66 (-0.3 mm): HousingFaceInput:1 ↔ 27mm_SandedScrew:17
- Mate:380: HousingFaceInput:1 ↔ 27mm_SandedScrew:17
- Flush:67 (-0.3 mm): HousingFaceInput:1 ↔ 27mm_SandedScrew:18
- Mate:381: HousingFaceInput:1 ↔ 27mm_SandedScrew:18
## Named parameters: d20_d4 = 0 mm, d21_d5 = 0 mm, d22_d6 = 0 mm, d23_d7 = 0 mm, d145_d2 = 0 mm, d146_d3 = 0 mm, d147_d4 = 0 mm, d148_d5 = 0 mm, d149_d131 = 0 mm, d150_d132 = 0 mm, d151_d6 = 0 mm, d152_d7 = 0 mm, d155_d2 = 0 mm, d156_d3 = 0 mm, d157_d4 = 0 mm, d158_d5 = 0 mm, d159_d131 = 0 mm, d160_d132 = 0 mm, d161_d6 = 0 mm, d162_d7 = 0 mm, d163_d155_d2 = 0 mm, d164_d156_d3 = 0 mm, d165_d157_d4 = 0 mm, d166_d158_d5 = 0 mm, d167_d159_d131 = 0 mm, d168_d160_d132 = 0 mm, d169_d161_d6 = 0 mm, d170_d162_d7 = 0 mm, d247_d2 = 0 mm, d248_d3 = 0 mm, d249_d4 = 0 mm, d250_d5 = 0 mm, d251_d131 = 0 mm, d252_d132 = 0 mm, d253_d6 = 0 mm, d254_d7 = 0 mm, d255_d247_d2 = 0 mm, d256_d248_d3 = 0 mm, d257_d249_d4 = 0 mm, d258_d250_d5 = 0 mm, d259_d251_d131 = 0 mm, d260_d252_d132 = 0 mm, d261_d253_d6 = 0 mm, d262_d254_d7 = 0 mm, d263_d247_d2 = 0 mm, d264_d248_d3 = 0 mm, d265_d249_d4 = 0 mm, d266_d250_d5 = 0 mm, d267_d251_d131 = 0 mm, d268_d252_d132 = 0 mm, d269_d253_d6 = 0 mm, d270_d254_d7 = 0 mm, d271_d247_d2 = 0 mm, d272_d248_d3 = 0 mm, d273_d249_d4 = 0 mm, d274_d250_d5 = 0 mm, d275_d251_d131 = 0 mm, d276_d252_d132 = 0 mm, d277_d253_d6 = 0 mm, d278_d254_d7 = 0 mm, d279_d247_d2 = 0 mm, d280_d248_d3 = 0 mm, d281_d249_d4 = 0 mm, d282_d250_d5 = 0 mm, d283_d251_d131 = 0 mm, d284_d252_d132 = 0 mm, d285_d253_d6 = 0 mm, d286_d254_d7 = 0 mm, d287_d247_d2 = 0 mm, d288_d248_d3 = 0 mm, d289_d249_d4 = 0 mm, d290_d250_d5 = 0 mm, d291_d251_d131 = 0 mm, d292_d252_d132 = 0 mm, d293_d253_d6 = 0 mm, d294_d254_d7 = 0 mm, d295_d247_d2 = 0 mm, d296_d248_d3 = 0 mm, d297_d249_d4 = 0 mm, d298_d250_d5 = 0 mm, d299_d251_d131 = 0 mm, d300_d252_d132 = 0 mm, d301_d253_d6 = 0 mm, d302_d254_d7 = 0 mm, d303_d247_d2 = 0 mm, d304_d248_d3 = 0 mm, d305_d249_d4 = 0 mm, d306_d250_d5 = 0 mm, d307_d251_d131 = 0 mm, d308_d252_d132 = 0 mm, d309_d253_d6 = 0 mm, d310_d254_d7 = 0 mm, d311_d247_d2 = 0 mm, d312_d248_d3 = 0 mm, d313_d249_d4 = 0 mm, d314_d250_d5 = 0 mm, d315_d251_d131 = 0 mm, d316_d252_d132 = 0 mm, d317_d253_d6 = 0 mm, d318_d254_d7 = 0 mm, d319_d247_d2 = 0 mm, d320_d248_d3 = 0 mm, d321_d249_d4 = 0 mm, d322_d250_d5 = 0 mm, d323_d251_d131 = 0 mm, d324_d252_d132 = 0 mm, d325_d253_d6 = 0 mm, d326_d254_d7 = 0 mm, d357_d247_d2 = 0 mm, d358_d248_d3 = 0 mm, d359_d249_d4 = 0 mm, d360_d250_d5 = 0 mm, d361_d251_d131 = 0 mm, d362_d252_d132 = 0 mm, d363_d253_d6 = 0 mm, d364_d254_d7 = 0 mm, d367_d247_d2 = 0 mm, d368_d248_d3 = 0 mm, d369_d249_d4 = 0 mm, d370_d250_d5 = 0 mm, d371_d251_d131 = 0 mm, d372_d252_d132 = 0 mm, d373_d253_d6 = 0 mm, d374_d254_d7 = 0 mm, d420_d319_d247_d2 = 0 mm, d421_d320_d248_d3 = 0 mm, d422_d321_d249_d4 = 0 mm, d423_d322_d250_d5 = 0 mm, d424_d323_d251_d131 = 0 mm, d425_d324_d252_d132 = 0 mm, d426_d325_d253_d6 = 0 mm, d427_d326_d254_d7 = 0 mm
